# Autodesk Inventor assembly: AutotunerCAD
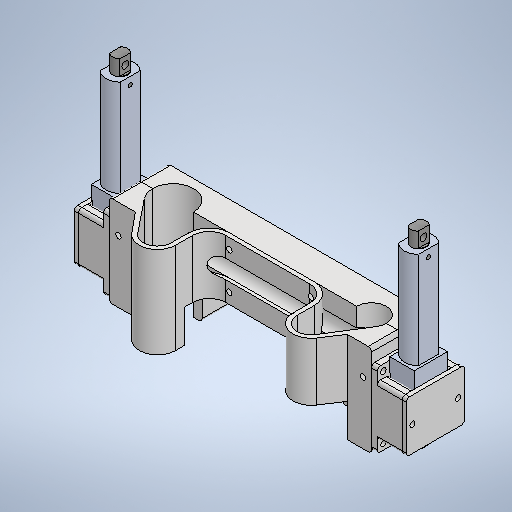
[picture p0: Inventor's stored thumbnail of the model, 512x512]
Saved by Autodesk Inventor 2026 (Build 300175050, 175E)
## iProperties
Created: 2025-12-10
Part Number: AutotunerCAD
Document SubType Name: Assembly
Designer: Nicholas M
Author: Nicholas M
## Documents named in this file (6)
- C:\Users\nmari\OneDrive\Desktop\Trombone-Autotuner\AutotunerCAD.iam
- C:\Users\nmari\OneDrive\Desktop\Trombone-Autotuner\BottomHalf2.ipt
- C:\Users\nmari\OneDrive\Desktop\Trombone-Autotuner\BottomHalf1.ipt
- C:\Users\nmari\OneDrive\Desktop\Trombone-Autotuner\MotorMount.ipt
- J:\Shared drives\Robot Ops -- CAD\Preseason 2025\Group 2\Drivetrain\Gearboxes\FIT0805.ipt
- C:\Users\nmari\OneDrive\Desktop\Trombone-Autotuner\BottomMountTop.ipt
## Components (8 placed, 5 different names)
1. BottomHalf1:1 — Mate:1, Mate:2, Flush:1, Mate:3, Mate:17, Mate:21
2. BottomHalf2:1 — Mate:1, Mate:2, Flush:1, Mate:16, Mate:19, Mate:20
3. MotorMount:1 — Mate:3, Mate:11, Mate:12, Angle:2, Mate:14, Mate:15, Mate:16, Mate:17, Mate:18
4. MotorMount:2 — Mate:9, Mate:10, Angle:1, Mate:19, Mate:20, Mate:21, Mate:22, Mate:23, Mate:24
5. FIT0805:1 — Mate:9, Mate:10, Angle:1
6. FIT0805:2 — Mate:11, Mate:12, Angle:2
7. BottomMountTop:1 — Mate:14, Mate:15, Mate:18
8. BottomMountTop:2 — Mate:22, Mate:23, Mate:24
## Relationships (21: Mate 18, Angle 2, Flush 1)
- Mate:1: BottomHalf1:1 ↔ BottomHalf2:1
- Mate:2: BottomHalf1:1 ↔ BottomHalf2:1
- Flush:1: BottomHalf1:1 ↔ BottomHalf2:1
- Mate:3: BottomHalf1:1 ↔ MotorMount:1
- Mate:9: MotorMount:2 ↔ FIT0805:1
- Mate:10: MotorMount:2 ↔ FIT0805:1
- Angle:1 (180 deg): MotorMount:2 ↔ FIT0805:1
- Mate:11: MotorMount:1 ↔ FIT0805:2
- Mate:12: MotorMount:1 ↔ FIT0805:2
- Angle:2 (180 deg): MotorMount:1 ↔ FIT0805:2
- Mate:14: MotorMount:1 ↔ BottomMountTop:1
- Mate:15: MotorMount:1 ↔ BottomMountTop:1
- Mate:16: BottomHalf2:1 ↔ MotorMount:1
- Mate:17: BottomHalf1:1 ↔ MotorMount:1
- Mate:18: MotorMount:1 ↔ BottomMountTop:1
- Mate:19: BottomHalf2:1 ↔ MotorMount:2
- Mate:20: BottomHalf2:1 ↔ MotorMount:2
- Mate:21: BottomHalf1:1 ↔ MotorMount:2
- Mate:22: MotorMount:2 ↔ BottomMountTop:2
- Mate:23: MotorMount:2 ↔ BottomMountTop:2
- Mate:24: MotorMount:2 ↔ BottomMountTop:2
